# Autodesk Inventor assembly: Left_Arm
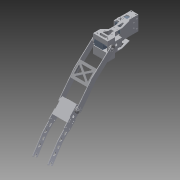
[picture p0: Inventor's stored thumbnail of the model, 180x180]
Saved by Autodesk Inventor 2013 (Build 170138000, 138)
## iProperties
Created: 2014-05-07
Part Number: Left_Arm
Document SubType Name: Assembly
Designer: andou
Mass: 431.276 g
Surface Area: 1646.92 cm^2
Volume: 241.289 cm^3
Density: 1.78738 g/cm^3
Author: andou
## Documents named in this file (17)
- C:\Users\andou\Documents\Inventor\RoboticsProject\project_4\Robot\Arm\Left_Arm\Left_Arm.iam
- C:\Users\andou\Documents\Inventor\RoboticsProject\project_4\Robot\All Common\Serial_Case.ipt
- C:\Users\andou\Documents\Inventor\RoboticsProject\project_4\Robot\All Common\KRS-2542HV.ipt
- C:\Users\andou\Documents\Inventor\RoboticsProject\project_4\Robot\Free_Horn\Free_Horn.iam
- C:\Users\andou\Documents\Inventor\RoboticsProject\project_4\Robot\All Common\Low_Height_Horn.ipt
- C:\Users\andou\Documents\Inventor\RoboticsProject\project_4\Robot\All Common\Horn_Spacer.ipt
- C:\Users\andou\Documents\Inventor\RoboticsProject\project_4\Robot\All Common\Washer(M4).ipt
- C:\Users\andou\Documents\Inventor\RoboticsProject\project_4\Robot\All Common\Nylon_Nat(M4).ipt
- C:\Users\andou\Documents\Inventor\RoboticsProject\project_4\Robot\All Common\Cap(M4-15).ipt
- C:\Users\andou\Documents\Inventor\RoboticsProject\project_4\Robot\All Common\Cap(M3-6).ipt
- C:\Users\andou\Documents\Inventor\RoboticsProject\project_4\Robot\Arm\Pitch_Serial_Case.ipt
- C:\Users\andou\Documents\Inventor\RoboticsProject\project_4\Robot\Arm\Arm_MiniLink.ipt
- C:\Users\andou\Documents\Inventor\RoboticsProject\project_4\Robot\Arm\Arm_MiniLink_Shim.ipt
- C:\Users\andou\Documents\Inventor\RoboticsProject\project_4\Robot\Arm\Yaw_Serial_Case.ipt
- C:\Users\andou\Documents\Inventor\RoboticsProject\project_4\Robot\Arm\Link_Supporter.ipt
- C:\Users\andou\Documents\Inventor\RoboticsProject\project_4\Robot\Arm\Arm_Link 120.ipt
- C:\Users\andou\Documents\Inventor\RoboticsProject\project_4\Robot\Arm\Arm_Link2.ipt
## Components (37 placed, 16 different names)
1. Free_Horn:1 [sub-assembly] — 挿入:15, 挿入:124, 挿入:137, 挿入:138
2. KRS-2542HV:1 — 挿入:8, 挿入:109, 挿入:110
3. Low_Height_Horn:1 — 挿入:8, 挿入:11, 挿入:12
4. Horn_Spacer:1 — 挿入:11, 挿入:12, 挿入:16, 挿入:139, 挿入:140
5. Washer(M4):1 — 挿入:14, 挿入:111
6. Nylon_Nat(M4):1 — 挿入:14
7. Cap(M4-15):1 — 挿入:15
8. Cap(M3-6):1 — 挿入:16
9. KRS-2542HV:2 — 挿入:25, 挿入:131, 挿入:132
10. Horn_Spacer:2 — 挿入:21, 挿入:23, 挿入:26, 挿入:165, 挿入:166
11. Free_Horn:2 [sub-assembly] — 挿入:114, 挿入:142, 挿入:169, 挿入:170
12. Cap(M3-6):2 — 挿入:23
13. Cap(M4-15):2 — 挿入:114
14. Low_Height_Horn:2 — 挿入:21, 挿入:25, 挿入:26
15. Washer(M4):2 — 挿入:22, 挿入:141
16. Nylon_Nat(M4):2 — 挿入:22
17. Serial_Case:3 — 挿入:33, 挿入:34, 挿入:37, 挿入:38, 挿入:174, 挿入:175, 挿入:176, 挿入:177
18. Nylon_Nat(M4):3 — 挿入:36
19. Washer(M4):3 — 挿入:36, 挿入:37
20. Low_Height_Horn:3 — 挿入:31, 挿入:32
21. Cap(M4-15):3 — 挿入:35
22. Cap(M3-6):3 — 挿入:39
23. Free_Horn:3 [sub-assembly] — 挿入:35, 挿入:38, 挿入:171
24. Horn_Spacer:3 — 挿入:31, 挿入:39, 挿入:172, 挿入:173
25. KRS-2542HV:3 — 挿入:32, 挿入:33, 挿入:34
26. Pitch_Serial_Case:1 — 挿入:109, 挿入:110, 挿入:111, 挿入:124
27. Arm_MiniLink:1 — 挿入:126, 挿入:130, 挿入:137, 挿入:138
28. Arm_MiniLink:2 — 挿入:125, 挿入:128, 挿入:139, 挿入:140
29. Arm_MiniLink_Shim:1 — 挿入:125, 挿入:128, 挿入:180, 挿入:181
30. Arm_MiniLink_Shim:2 — 挿入:126, 挿入:130, 挿入:178, 挿入:179
31. Arm_MiniLink_Shim:3 — 挿入:178, 挿入:179, 挿入:182, 挿入:183
32. Yaw_Serial_Case:1 — 挿入:131, 挿入:132, 挿入:141, 挿入:142, 挿入:180, 挿入:181, 挿入:182, 挿入:183
33. Link_Supporter:1 — 挿入:167, 挿入:168
34. Arm_Link 120:1 — 挿入:174, 挿入:175
35. Arm_Link 120:2 — 挿入:176, 挿入:177
36. Arm_Link2:1 — 挿入:169, 挿入:170, 挿入:171
37. Arm_Link2:2 — 挿入:165, 挿入:166, 挿入:167, 挿入:168, 挿入:172, 挿入:173
## Relationships (56: Insert 56)
- 挿入:8 [Insert]: KRS-2542HV:1 ↔ Low_Height_Horn:1
- 挿入:11 [Insert]: Low_Height_Horn:1 ↔ Horn_Spacer:1
- 挿入:12 [Insert]: Low_Height_Horn:1 ↔ Horn_Spacer:1
- 挿入:14 [Insert]: Washer(M4):1 ↔ Nylon_Nat(M4):1
- 挿入:15 [Insert]: Free_Horn:1 ↔ Cap(M4-15):1
- 挿入:16 [Insert]: Horn_Spacer:1 ↔ Cap(M3-6):1
- 挿入:21 [Insert]: Horn_Spacer:2 ↔ Low_Height_Horn:2
- 挿入:22 [Insert]: Washer(M4):2 ↔ Nylon_Nat(M4):2
- 挿入:23 [Insert]: Horn_Spacer:2 ↔ Cap(M3-6):2
- 挿入:25 [Insert]: KRS-2542HV:2 ↔ Low_Height_Horn:2
- 挿入:26 [Insert]: Horn_Spacer:2 ↔ Low_Height_Horn:2
- 挿入:31 [Insert]: Low_Height_Horn:3 ↔ Horn_Spacer:3
- 挿入:32 [Insert]: Low_Height_Horn:3 ↔ KRS-2542HV:3
- 挿入:33 [Insert]: Serial_Case:3 ↔ KRS-2542HV:3
- 挿入:34 [Insert]: Serial_Case:3 ↔ KRS-2542HV:3
- 挿入:35 [Insert]: Cap(M4-15):3 ↔ Free_Horn:3
- 挿入:36 [Insert]: Nylon_Nat(M4):3 ↔ Washer(M4):3
- 挿入:37 [Insert]: Serial_Case:3 ↔ Washer(M4):3
- 挿入:38 [Insert]: Serial_Case:3 ↔ Free_Horn:3
- 挿入:39 [Insert]: Cap(M3-6):3 ↔ Horn_Spacer:3
- 挿入:109 [Insert]: KRS-2542HV:1 ↔ Pitch_Serial_Case:1
- 挿入:110 [Insert]: KRS-2542HV:1 ↔ Pitch_Serial_Case:1
- 挿入:111 [Insert]: Washer(M4):1 ↔ Pitch_Serial_Case:1
- 挿入:114 [Insert]: Free_Horn:2 ↔ Cap(M4-15):2
- 挿入:124 [Insert]: Free_Horn:1 ↔ Pitch_Serial_Case:1
- 挿入:125 [Insert]: Arm_MiniLink:2 ↔ Arm_MiniLink_Shim:1
- 挿入:126 [Insert]: Arm_MiniLink:1 ↔ Arm_MiniLink_Shim:2
- 挿入:128 [Insert]: Arm_MiniLink:2 ↔ Arm_MiniLink_Shim:1
- 挿入:130 [Insert]: Arm_MiniLink:1 ↔ Arm_MiniLink_Shim:2
- 挿入:131 [Insert]: KRS-2542HV:2 ↔ Yaw_Serial_Case:1
- 挿入:132 [Insert]: KRS-2542HV:2 ↔ Yaw_Serial_Case:1
- 挿入:137 [Insert]: Free_Horn:1 ↔ Arm_MiniLink:1
- 挿入:138 [Insert]: Free_Horn:1 ↔ Arm_MiniLink:1
- 挿入:139 [Insert]: Horn_Spacer:1 ↔ Arm_MiniLink:2
- 挿入:140 [Insert]: Horn_Spacer:1 ↔ Arm_MiniLink:2
- 挿入:141 [Insert]: Washer(M4):2 ↔ Yaw_Serial_Case:1
- 挿入:142 [Insert]: Free_Horn:2 ↔ Yaw_Serial_Case:1
- 挿入:165 [Insert]: Horn_Spacer:2 ↔ Arm_Link2:2
- 挿入:166 [Insert]: Horn_Spacer:2 ↔ Arm_Link2:2
- 挿入:167 [Insert]: Link_Supporter:1 ↔ Arm_Link2:2
- 挿入:168 [Insert]: Link_Supporter:1 ↔ Arm_Link2:2
- 挿入:169 [Insert]: Free_Horn:2 ↔ Arm_Link2:1
- 挿入:170 [Insert]: Free_Horn:2 ↔ Arm_Link2:1
- 挿入:171 [Insert]: Free_Horn:3 ↔ Arm_Link2:1
- 挿入:172 [Insert]: Horn_Spacer:3 ↔ Arm_Link2:2
- 挿入:173 [Insert]: Horn_Spacer:3 ↔ Arm_Link2:2
- 挿入:174 [Insert]: Serial_Case:3 ↔ Arm_Link 120:1
- 挿入:175 [Insert]: Serial_Case:3 ↔ Arm_Link 120:1
- 挿入:176 [Insert]: Serial_Case:3 ↔ Arm_Link 120:2
- 挿入:177 [Insert]: Serial_Case:3 ↔ Arm_Link 120:2
- 挿入:178 [Insert]: Arm_MiniLink_Shim:2 ↔ Arm_MiniLink_Shim:3
- 挿入:179 [Insert]: Arm_MiniLink_Shim:2 ↔ Arm_MiniLink_Shim:3
- 挿入:180 [Insert]: Arm_MiniLink_Shim:1 ↔ Yaw_Serial_Case:1
- 挿入:181 [Insert]: Arm_MiniLink_Shim:1 ↔ Yaw_Serial_Case:1
- 挿入:182 [Insert]: Arm_MiniLink_Shim:3 ↔ Yaw_Serial_Case:1
- 挿入:183 [Insert]: Arm_MiniLink_Shim:3 ↔ Yaw_Serial_Case:1
## Named parameters: sa_0 = 99.9999, sa_1 = -0.136179, sa_2 = -5.34164e-05
note: some values were not read from the file. Shown as the stored number, unit unknown: "sa_0", "sa_1", "sa_2".
